# Autodesk Inventor assembly: Final Leg Assembly
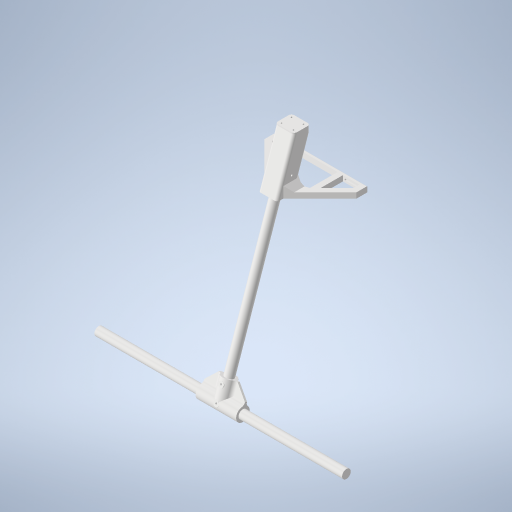
[picture p0: Inventor's stored thumbnail of the model, 512x512]
Saved by Autodesk Inventor 2023 (Build 270158000, 158)
## iProperties
Created: 2023-01-18
Part Number: Final Leg Assembly
Document SubType Name: Assembly
Designer: chase
Author: chase
## Documents named in this file (5)
- C:\Users\Administrator\Documents\GitHub\WU-Team20-AutonomousDrone\CAD\Legs\Final Leg Assembly.iam
- C:\Users\Administrator\Documents\GitHub\WU-Team20-AutonomousDrone\CAD\Raw Models\CarbonTube-16mmOD.ipt
- C:\Users\Administrator\Documents\GitHub\WU-Team20-AutonomousDrone\CAD\Legs\LegTeeJoint2.5.ipt
- C:\Users\Administrator\Documents\GitHub\WU-Team20-AutonomousDrone\CAD\Legs\Landing Foot.ipt
- C:\Users\Administrator\Documents\GitHub\WU-Team20-AutonomousDrone\CAD\Legs\UpperLandingLegMount WebBrace+Shortened.ipt
## Components (4 placed, 4 different names)
1. CarbonTube-16mmOD:1 — Insert:2, Rigid:1
2. LegTeeJoint2.5:1 — Insert:2, Insert:3
3. Landing Foot:1 — Insert:3
4. UpperLandingLegMount WebBrace+Shortened:1 — Rigid:1
## Relationships (3: Insert 2, WeldJoint 1)
- Insert:2: CarbonTube-16mmOD:1 ↔ LegTeeJoint2.5:1
- Insert:3 (-191.1 mm): LegTeeJoint2.5:1 ↔ Landing Foot:1
- Rigid:1 [WeldJoint]: CarbonTube-16mmOD:1 ↔ UpperLandingLegMount WebBrace+Shortened:1
